# Autodesk Inventor assembly: 部件1
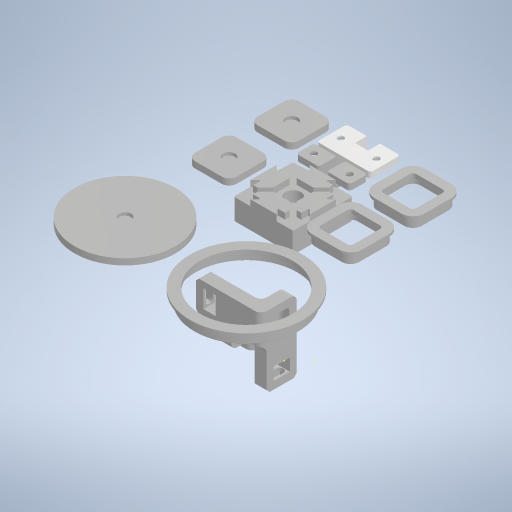
[picture p0: Inventor's stored thumbnail of the model, 512x512]
Saved by Autodesk Inventor 2024 (Build 280153000, 153)
## iProperties
Created: 2023-06-19
Part Number: 部件1
Document SubType Name: Assembly
Designer: lunima
Author: lunima
## Documents named in this file (6)
- C:\Users\lunima\Desktop\DOSYN\部件1.iam
- C:\Users\lunima\Desktop\DOSYN\IPT\LED Cover\LED Cover Cable Strain Relief Clip.ipt
- C:\Users\lunima\Desktop\DOSYN\IPT\LED Cover\LED Cover Drag Chain Termination.ipt
- C:\Users\lunima\Desktop\DOSYN\IPT\Main Structure\Side Lid.ipt
- C:\Users\lunima\Desktop\DOSYN\小零件组合.iam
- C:\Users\lunima\Desktop\DOSYN\IPT\Carriage\Pogo Pin Clip.ipt
## Components (5 placed, 5 different names)
1. LED Cover Cable Strain Relief Clip:1 — 配合:1, 表面齐平:1, 表面齐平:2, 表面齐平:3, 配合:2, 表面齐平:4
2. LED Cover Drag Chain Termination:1 — 配合:1, 表面齐平:1, 表面齐平:2, 表面齐平:6
3. Side Lid:1 — 表面齐平:3, 配合:2, 表面齐平:4, 表面齐平:5
4. 小零件组合:1 [sub-assembly] — 表面齐平:5, 表面齐平:6, 表面齐平:7
5. Pogo Pin Clip:1 — 表面齐平:7
## Relationships (9: Flush 7, Mate 2)
- 配合:1 [Mate] (1 mm): LED Cover Cable Strain Relief Clip:1 ↔ LED Cover Drag Chain Termination:1
- 表面齐平:1 [Flush]: LED Cover Cable Strain Relief Clip:1 ↔ LED Cover Drag Chain Termination:1
- 表面齐平:2 [Flush]: LED Cover Cable Strain Relief Clip:1 ↔ LED Cover Drag Chain Termination:1
- 表面齐平:3 [Flush]: LED Cover Cable Strain Relief Clip:1 ↔ Side Lid:1
- 配合:2 [Mate] (1 mm): LED Cover Cable Strain Relief Clip:1 ↔ Side Lid:1
- 表面齐平:4 [Flush]: LED Cover Cable Strain Relief Clip:1 ↔ Side Lid:1
- 表面齐平:5 [Flush]: Side Lid:1 ↔ 小零件组合:1
- 表面齐平:6 [Flush]: LED Cover Drag Chain Termination:1 ↔ 小零件组合:1
- 表面齐平:7 [Flush]: 小零件组合:1 ↔ Pogo Pin Clip:1
